# Autodesk Inventor assembly: Stanina
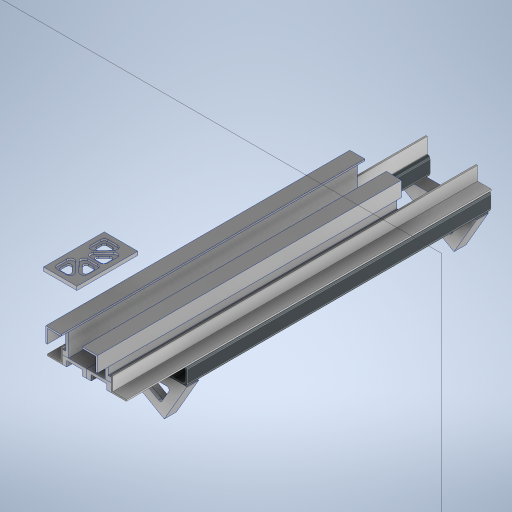
[picture p0: Inventor's stored thumbnail of the model, 512x512]
Saved by Autodesk Inventor 2024 (Build 280153000, 153)
## iProperties
Created: 2023-08-15
Part Number: Stanina
Document SubType Name: Assembly
Designer: Kippi
Mass: 37121.2 g
Surface Area: 30256.4 cm^2
Volume: 10840.5 cm^3
Density: 3.42432 g/cm^3
Author: Kippi
## Documents named in this file (9)
- C:\WorkProject\CNC_Lathe\Stanina.iam
- C:\WorkProject\CNC_Lathe\L_PlNKA800.ipt
- C:\WorkProject\CNC_Lathe\Ugol800.ipt
- C:\WorkProject\CNC_Lathe\L_PlNKA_Niz.ipt
- C:\WorkProject\CNC_Lathe\PlaskaUkrep.ipt
- C:\WorkProject\CNC_Lathe\Truba60.ipt
- C:\WorkProject\CNC_Lathe\Ugol1300.ipt
- C:\WorkProject\CNC_Lathe\StaninaOpora.iam.ipt
- StaninaOpora.iam
## Components (13 placed, 7 different names)
1. L_PlNKA_Niz:1 — Mate:1, Flush:1, Flush:2, Mate:8, Mate:16, Flush:18, Flush:19, Mate:20, Flush:24, Flush:26
2. L_PlNKA_Niz:2 — Mate:1, Flush:1, Flush:2, Mate:8, Mate:19, Flush:25, Flush:27
3. L_PlNKA800:3 — Mate:27, Mate:28, Flush:35
4. L_PlNKA800:4 — Mate:16, Flush:18, Flush:19, Mate:25, Mate:26, Flush:34
5. Ugol1300:1 — Mate:19, Flush:25, Flush:27, Mate:22, Flush:30, Flush:31
6. Truba60:3 — Mate:22, Flush:30, Flush:31, Mate:23, Mate:24, Flush:32
7. Truba60:4 — Mate:21, Flush:28, Flush:29
8. Ugol1300:3 — Mate:20, Flush:24, Flush:26, Mate:21, Flush:28, Flush:29
9. StaninaOpora.iam:1 — Mate:23, Flush:33
10. StaninaOpora.iam:2 — Mate:24, Flush:32, Flush:33
11. Ugol800:3 — Mate:27, Mate:28, Flush:35
12. Ugol800:4 — Mate:25, Mate:26, Flush:34
13. PlaskaUkrep:3
## Relationships (29: Flush 16, Mate 13)
- Mate:1: L_PlNKA_Niz:1 ↔ L_PlNKA_Niz:2
- Flush:1: L_PlNKA_Niz:1 ↔ L_PlNKA_Niz:2
- Flush:2: L_PlNKA_Niz:1 ↔ L_PlNKA_Niz:2
- Mate:8: L_PlNKA_Niz:1 ↔ L_PlNKA_Niz:2
- Mate:16: L_PlNKA_Niz:1 ↔ L_PlNKA800:4
- Flush:18: L_PlNKA_Niz:1 ↔ L_PlNKA800:4
- Flush:19: L_PlNKA_Niz:1 ↔ L_PlNKA800:4
- Mate:19: L_PlNKA_Niz:2 ↔ Ugol1300:1
- Mate:20: L_PlNKA_Niz:1 ↔ Ugol1300:3
- Flush:24: L_PlNKA_Niz:1 ↔ Ugol1300:3
- Flush:25: L_PlNKA_Niz:2 ↔ Ugol1300:1
- Flush:26: L_PlNKA_Niz:1 ↔ Ugol1300:3
- Flush:27: L_PlNKA_Niz:2 ↔ Ugol1300:1
- Mate:21: Truba60:4 ↔ Ugol1300:3
- Flush:28: Truba60:4 ↔ Ugol1300:3
- Flush:29: Truba60:4 ↔ Ugol1300:3
- Mate:22: Ugol1300:1 ↔ Truba60:3
- Flush:30: Ugol1300:1 ↔ Truba60:3
- Flush:31: Ugol1300:1 ↔ Truba60:3
- Mate:23: Truba60:3 ↔ StaninaOpora.iam:1
- Mate:24: Truba60:3 ↔ StaninaOpora.iam:2
- Flush:32: Truba60:3 ↔ StaninaOpora.iam:2
- Flush:33: StaninaOpora.iam:1 ↔ StaninaOpora.iam:2
- Mate:25: L_PlNKA800:4 ↔ Ugol800:4
- Mate:26: L_PlNKA800:4 ↔ Ugol800:4
- Flush:34: L_PlNKA800:4 ↔ Ugol800:4
- Mate:27: L_PlNKA800:3 ↔ Ugol800:3
- Mate:28: L_PlNKA800:3 ↔ Ugol800:3
- Flush:35: L_PlNKA800:3 ↔ Ugol800:3
